# Autodesk Inventor assembly: Assembly2
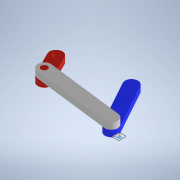
[picture p0: Inventor's stored thumbnail of the model, 180x180]
Saved by Autodesk Inventor 2022 (Build 260153000, 153)
## iProperties
Created: 2022-03-13
Part Number: Assembly2
Document SubType Name: Assembly
Designer: br4ch
Author: br4ch
## Documents named in this file (4)
- C:\Users\br4ch\M-and-Ms\Ansys labs\4 bar\Assembly2.iam
- C:\Users\br4ch\M-and-Ms\Ansys labs\4 bar\Part1.ipt
- C:\Users\br4ch\M-and-Ms\Ansys labs\4 bar\Part2.ipt
- C:\Users\br4ch\M-and-Ms\Ansys labs\4 bar\Part4.ipt
## Components (3 placed, 3 different names)
1. Part1:1 — Rotational:9
2. Part2:1 — Rotational:8, Rotational:9
3. Part4:1 — Rotational:8
## Relationships (2: RevoluteJoint 2)
- Rotational:8 [RevoluteJoint]: Part2:1 ↔ Part4:1
- Rotational:9 [RevoluteJoint]: Part1:1 ↔ Part2:1
